# Autodesk Inventor assembly: CaseB
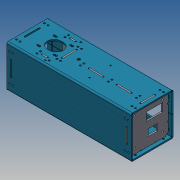
[picture p0: Inventor's stored thumbnail of the model, 180x180]
Saved by Autodesk Inventor 2017 (Build 210142000, 142)
## iProperties
Part Number: CaseB
Material: Genérico
Document SubType Name: Assembly
Designer: Leo
Author: Leo
## Documents named in this file (6)
- C:\Users\Leo\Dropbox\E\Caja Motriz\CaseB.iam
- C:\Users\Leo\Dropbox\E\Caja Motriz\Case\Protector.ipt
- C:\Users\Leo\Dropbox\E\Caja Motriz\Case\CaseB.ipt
- C:\Users\Leo\Dropbox\E\Caja Motriz\Case\Refuerzo U.ipt
- C:\Users\Leo\Dropbox\E\Caja Motriz\Case\bandeja central.ipt
- C:\Users\Leo\Dropbox\E\Caja Motriz\Case\Tapa Enchufes.ipt
## Components (5 placed, 5 different names)
1. CaseB:1 — Coincidencia:1, Nivelación:5, Nivelación:6, Nivelación:7, Coincidencia:2, Nivelación:8, Nivelación:10
2. Protector:1 — Nivelación:1, Nivelación:2, Nivelación:3
3. Refuerzo U:1 — Nivelación:4, Coincidencia:1, Nivelación:5
4. bandeja central:1 — Nivelación:6, Nivelación:7, Coincidencia:2
5. Tapa Enchufes:1 — Nivelación:8, Nivelación:9, Nivelación:10
## Relationships (12: Flush 10, Mate 2)
- Nivelación:1 [Flush] (40 mm): Protector:1
- Nivelación:2 [Flush]: Protector:1
- Nivelación:3 [Flush]: Protector:1
- Nivelación:4 [Flush]: Refuerzo U:1
- Coincidencia:1 [Mate]: CaseB:1 ↔ Refuerzo U:1
- Nivelación:5 [Flush]: CaseB:1 ↔ Refuerzo U:1
- Nivelación:6 [Flush]: CaseB:1 ↔ bandeja central:1
- Nivelación:7 [Flush]: CaseB:1 ↔ bandeja central:1
- Coincidencia:2 [Mate]: CaseB:1 ↔ bandeja central:1
- Nivelación:8 [Flush]: CaseB:1 ↔ Tapa Enchufes:1
- Nivelación:9 [Flush]: Tapa Enchufes:1
- Nivelación:10 [Flush]: CaseB:1 ↔ Tapa Enchufes:1
